# Autodesk Inventor assembly: robot
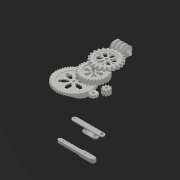
[picture p0: Inventor's stored thumbnail of the model, 180x180]
Saved by Autodesk Inventor 2020 (Build 240168000, 168)
## iProperties
Created: 2020-07-14
Part Number: robot
Document SubType Name: Assembly
Designer: alons
Author: alons
## Documents named in this file (10)
- C:\Users\alons\OneDrive\Documents\GitHub\Water-Strider-Robot\Striderbot\robot.iam
- C:\Users\alons\OneDrive\Documents\GitHub\Water-Strider-Robot\Striderbot\worm_gear_mesh_1\Design Accelerator\Worm14.ipt
- C:\Users\alons\OneDrive\Documents\GitHub\Water-Strider-Robot\Striderbot\worm_gear_mesh_1\Design Accelerator\Worm Gear14.ipt
- C:\Users\alons\OneDrive\Documents\GitHub\Water-Strider-Robot\Striderbot\spur_gears_mesh_2\Design Accelerator\Spur Gear13.ipt
- C:\Users\alons\OneDrive\Documents\GitHub\Water-Strider-Robot\Striderbot\spur_gears_mesh_2\Design Accelerator\Spur Gear23.ipt
- C:\Users\alons\OneDrive\Documents\GitHub\Water-Strider-Robot\Striderbot\spur_gears_mesh_3\Design Accelerator\Spur Gear11.ipt
- C:\Users\alons\OneDrive\Documents\GitHub\Water-Strider-Robot\Striderbot\spur_gears_mesh_3\Design Accelerator\Spur Gear21.ipt
- C:\Users\alons\OneDrive\Documents\GitHub\Water-Strider-Robot\Striderbot\Crank_Rocker\Link_1.ipt
- C:\Users\alons\OneDrive\Documents\GitHub\Water-Strider-Robot\Striderbot\Crank_Rocker\Link_2.ipt
- C:\Users\alons\OneDrive\Documents\GitHub\Water-Strider-Robot\Striderbot\Crank_Rocker\Link_3.ipt
## Components (9 placed, 7 different names)
1. Worm:1 — Mate:1, Mate:2, Flush:1, Tangent:1
2. Worm Gear:1 — Flush:1, Tangent:1, Mate:3, Mate:4
3. Spur Gear1:1 — Mate:4, Tangent:2
4. Spur Gear2:1 — Tangent:2, Mate:5
5. Spur Gear1:2 — Mate:5, Tangent:3
6. Spur Gear2:2 — Tangent:3
7. Link_1:1
8. Link_2:1
9. Link_3:1
## Relationships (9: Mate 5, Tangent 3, Flush 1)
- Mate:1: Worm:1
- Mate:2: Worm:1
- Flush:1: Worm:1 ↔ Worm Gear:1
- Tangent:1: Worm:1 ↔ Worm Gear:1
- Mate:3: Worm Gear:1
- Mate:4: Worm Gear:1 ↔ Spur Gear1:1
- Tangent:2: Spur Gear1:1 ↔ Spur Gear2:1
- Mate:5: Spur Gear2:1 ↔ Spur Gear1:2
- Tangent:3: Spur Gear1:2 ↔ Spur Gear2:2
